# Autodesk Inventor assembly: Motor
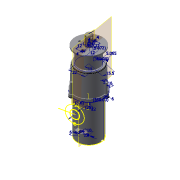
[picture p0: Inventor's stored thumbnail of the model, 180x180]
Saved by Autodesk Inventor 2015 SP1 (Build 190203100, 203)
## iProperties
Created: 2014-08-26
Part Number: Motor
Document SubType Name: Assembly
Designer: laca
Mass: 60.3175 g
Surface Area: 430.355 cm^2
Volume: 60.3175 cm^3
Density: 1 g/cm^3
Author: laca
## Documents named in this file (9)
- C:\Users\laca\Desktop\Allamvizsga\Invntor\RobotMechanikaForMAtlabVer2\Motor.iam
- C:\Users\laca\Desktop\Allamvizsga\Invntor\RobotMechanikaForMAtlabVer2\Haz.ipt
- C:\Users\laca\Desktop\Allamvizsga\Invntor\RobotMechanikaForMAtlabVer2\MotorFenek.ipt
- C:\Users\laca\Desktop\Allamvizsga\Invntor\RobotMechanikaForMAtlabVer2\Rotor.ipt
- C:\Users\laca\Desktop\Allamvizsga\Invntor\RobotMechanikaForMAtlabVer2\ReduktorLemez.ipt
- C:\Users\laca\Desktop\Allamvizsga\Invntor\RobotMechanikaForMAtlabVer2\ReduktorHaz.ipt
- C:\Users\laca\Desktop\Allamvizsga\Invntor\RobotMechanikaForMAtlabVer2\AlatetMotor.ipt
- C:\Users\laca\Desktop\Allamvizsga\Invntor\RobotMechanikaForMAtlabVer2\Tengely.ipt
- C:\Users\laca\Desktop\Allamvizsga\Invntor\RobotMechanikaForMAtlabVer2\KuplungZar.ipt
## Components (8 placed, 8 different names)
1. Haz:1 — Rotational:1, Insert:1, Insert:3, Insert:4, Insert:5, Mate:3
2. MotorFenek:1 — Mate:1, Rotational:1, Insert:5, Mate:3
3. Rotor:1 — Insert:1
4. ReduktorLemez:1 — Mate:2, Insert:2, Insert:3, Insert:4
5. ReduktorHaz:1 — Mate:2, Insert:2, Insert:6, Insert:7, Angle:1, Flush:1, Insert:9
6. AlatetMotor:1 — Insert:6, Insert:7, Insert:8
7. Tengely:1 — Insert:8, Tangent:1
8. KuplungZar:1 — Flush:1, Insert:9
## Relationships (16: Insert 9, Mate 3, RevoluteJoint 1, Angle 1, Tangent 1, Flush 1)
- Mate:1: MotorFenek:1
- Rotational:1 [RevoluteJoint]: Haz:1 ↔ MotorFenek:1
- Insert:1: Haz:1 ↔ Rotor:1
- Mate:2: ReduktorLemez:1 ↔ ReduktorHaz:1
- Insert:2: ReduktorLemez:1 ↔ ReduktorHaz:1
- Insert:3: Haz:1 ↔ ReduktorLemez:1
- Insert:4: Haz:1 ↔ ReduktorLemez:1
- Insert:5: Haz:1 ↔ MotorFenek:1
- Mate:3: Haz:1 ↔ MotorFenek:1
- Insert:6: ReduktorHaz:1 ↔ AlatetMotor:1
- Insert:7: ReduktorHaz:1 ↔ AlatetMotor:1
- Insert:8 (-2 mm): AlatetMotor:1 ↔ Tengely:1
- Angle:1 (0 deg): ReduktorHaz:1
- Tangent:1: Tengely:1
- Flush:1: ReduktorHaz:1 ↔ KuplungZar:1
- Insert:9: ReduktorHaz:1 ↔ KuplungZar:1
